# Autodesk Inventor assembly: OdometryAssembly
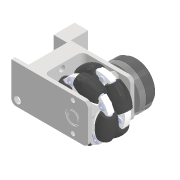
[picture p0: Inventor's stored thumbnail of the model, 180x180]
Saved by Autodesk Inventor 2020 (Build 240168000, 168)
## iProperties
Created: 2019-07-05
Part Number: OdometryAssembly
Document SubType Name: Assembly
Designer: ishaa
Author: ishaa
## Documents named in this file (9)
- D:\ishaa\Documents\GrabCAD\FTC\Part Files\Reusable Parts\GoBildaOdometry\OdometryAssembly.iam
- D:\ishaa\Documents\GrabCAD\FTC\Part Files\Reusable Parts\GoBildaOdometry\Odometry Holder.ipt
- D:\ishaa\Documents\GrabCAD\FTC\Part Files\US Digital\E8T-X-236-S-D-M-X.ipt
- D:\ishaa\Documents\GrabCAD\FTC\Part Files\Actobotics\All STEP Files\535 parts\535042.ipt
- D:\ishaa\Documents\GrabCAD\FTC\Part Files\Reusable Parts\ActoboticsOdometry\14166.iam
- D:\ishaa\Documents\GrabCAD\FTC\Part Files\Mcmaster\90576A161_MEDIUM-STRENGTH STEEL NYLON-INSERT LOCKNUT.ipt
- D:\ishaa\Documents\GrabCAD\FTC\Part Files\Reusable Parts\GoBildaOdometry\spacer.ipt
- D:\ishaa\Documents\GrabCAD\FTC\Part Files\Reusable Parts\GoBildaOdometry\spacerNutSide.ipt
- D:\ishaa\Documents\GrabCAD\FTC\Part Files\Actobotics\All STEP Files\634 parts\634064.ipt
## Components (10 placed, 8 different names)
1. Odometry Holder:1 — Insert:1, Mate:1, Insert:2, Insert:3, Insert:4, Insert:5, Flush:1
2. E8T-X-236-S-D-M-X:1 — Insert:1, Mate:1
3. 535042:1 — Insert:2, Insert:6
4. 535042:2 — Insert:3, Mate:2, Insert:7, Mate:4
5. 14166:1 [sub-assembly] — Mate:2, Mate:3
6. 90576A161_MEDIUM-STRENGTH STEEL NYLON-INSERT LOCKNUT:1 — Insert:4
7. 90576A161_MEDIUM-STRENGTH STEEL NYLON-INSERT LOCKNUT:2 — Insert:5
8. spacer:1 — Insert:6, Mate:3
9. spacerNutSide:1 — Insert:7
10. 634064:1 — Mate:4, Flush:1
## Relationships (12: Insert 7, Mate 4, Flush 1)
- Insert:1: Odometry Holder:1 ↔ E8T-X-236-S-D-M-X:1
- Mate:1: Odometry Holder:1 ↔ E8T-X-236-S-D-M-X:1
- Insert:2: Odometry Holder:1 ↔ 535042:1
- Insert:3: Odometry Holder:1 ↔ 535042:2
- Mate:2: 535042:2 ↔ 14166:1
- Insert:4: Odometry Holder:1 ↔ 90576A161_MEDIUM-STRENGTH STEEL NYLON-INSERT LOCKNUT:1
- Insert:5: Odometry Holder:1 ↔ 90576A161_MEDIUM-STRENGTH STEEL NYLON-INSERT LOCKNUT:2
- Insert:6: 535042:1 ↔ spacer:1
- Mate:3: 14166:1 ↔ spacer:1
- Insert:7: 535042:2 ↔ spacerNutSide:1
- Mate:4: 535042:2 ↔ 634064:1
- Flush:1: Odometry Holder:1 ↔ 634064:1
